# Autodesk Inventor assembly: Link_01_Assembly
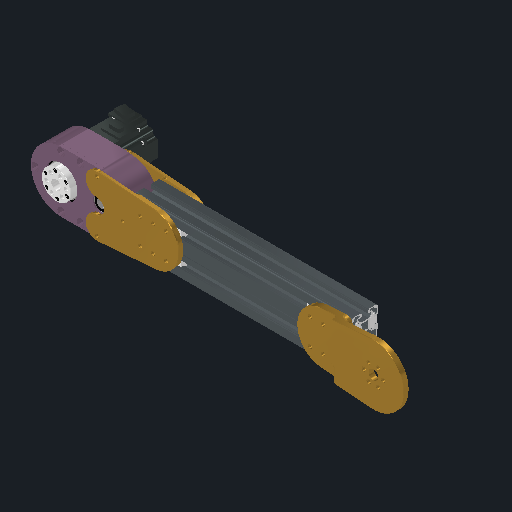
[picture p0: Inventor's stored thumbnail of the model, 512x512]
Saved by Autodesk Inventor 2026 (Build 300175000, 175)
## iProperties
Created: 2025-11-30
Part Number: Link_01_Assembly
Document SubType Name: Assembly
Designer: pochi
Mass: 2645.35 g
Surface Area: 5783.73 cm^2
Volume: 1224.73 cm^3
Density: 2.15995 g/cm^3
Author: pochi
## Documents named in this file (5)
- D:\POLIMI\3RD SEMESTER\Industrial Robotics\Project\Mine\Link_01_Assembly.iam
- D:\POLIMI\3RD SEMESTER\Industrial Robotics\Project\Mine\Link_01.ipt
- D:\POLIMI\3RD SEMESTER\Industrial Robotics\Project\Mine\RigidConector_40x80.ipt
- D:\POLIMI\3RD SEMESTER\Industrial Robotics\Project\Mine\RotationalConector_40x80.ipt
- D:\POLIMI\3RD SEMESTER\Industrial Robotics\Project\Mine\Reducer.iam
## Components (5 placed, 4 different names)
1. Link_01:1 — Mate:1, Mate:2, Mate:3, Mate:4, Mate:5, Mate:6, Mate:7, Mate:8, Mate:9
2. RigidConector_40x80:1 — Mate:1, Mate:2, Mate:3, Mate:11, Mate:12
3. RigidConector_40x80:2 — Mate:4, Mate:5, Mate:6, Mate:10
4. RotationalConector_40x80:1 — Mate:7, Mate:8, Mate:9
5. Reducer:1 [sub-assembly] — Mate:10, Mate:11, Mate:12
## Relationships (12: Mate 12)
- Mate:1: Link_01:1 ↔ RigidConector_40x80:1
- Mate:2: Link_01:1 ↔ RigidConector_40x80:1
- Mate:3: Link_01:1 ↔ RigidConector_40x80:1
- Mate:4: Link_01:1 ↔ RigidConector_40x80:2
- Mate:5: Link_01:1 ↔ RigidConector_40x80:2
- Mate:6: Link_01:1 ↔ RigidConector_40x80:2
- Mate:7: Link_01:1 ↔ RotationalConector_40x80:1
- Mate:8: Link_01:1 ↔ RotationalConector_40x80:1
- Mate:9: Link_01:1 ↔ RotationalConector_40x80:1
- Mate:10: RigidConector_40x80:2 ↔ Reducer:1
- Mate:11: RigidConector_40x80:1 ↔ Reducer:1
- Mate:12: RigidConector_40x80:1 ↔ Reducer:1
